# Autodesk Inventor assembly: Assembly
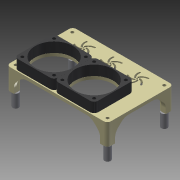
[picture p0: Inventor's stored thumbnail of the model, 180x180]
Saved by Autodesk Inventor 2014 (Build 180170000, 170)
## iProperties
Created: 2017-03-01
Part Number: Assembly
Document SubType Name: Assembly
Designer: Rubén
Author: Rubén
## Documents named in this file (4)
- C:\Users\Rubén\Documents\GitHub\my-3D-printing-designs\Prusa i3 Steel parts\SAV case\Version #2\Assembly.iam
- C:\Users\Rubén\Documents\GitHub\my-3D-printing-designs\Prusa i3 Steel parts\SAV case\Version #2\SAV case.ipt
- C:\Users\Rubén\Documents\GitHub\my-3D-printing-designs\Prusa i3 Steel parts\SAV case\Version #2\Fan 4x4.ipt
- C:\Users\Rubén\Documents\GitHub\my-3D-printing-designs\Prusa i3 Steel parts\SAV case\Version #2\SAV separator.ipt
## Components (7 placed, 3 different names)
1. SAV case:1 — Mate:1, Mate:2, Mate:3, Mate:4, Mate:5, Mate:6, Mate:7, Mate:8, Mate:9, Mate:10, Mate:11, Mate:12, Mate:13, Mate:14
2. Fan 4x4:1 — Mate:4, Mate:5, Mate:6
3. Fan 4x4:2 — Mate:1, Mate:2, Mate:3
4. SAV separator:1 — Mate:7, Mate:11
5. SAV separator:2 — Mate:9, Mate:13
6. SAV separator:3 — Mate:8, Mate:14
7. SAV separator:4 — Mate:10, Mate:12
## Relationships (14: Mate 14)
- Mate:1: SAV case:1 ↔ Fan 4x4:2
- Mate:2: SAV case:1 ↔ Fan 4x4:2
- Mate:3: SAV case:1 ↔ Fan 4x4:2
- Mate:4: SAV case:1 ↔ Fan 4x4:1
- Mate:5: SAV case:1 ↔ Fan 4x4:1
- Mate:6: SAV case:1 ↔ Fan 4x4:1
- Mate:7: SAV case:1 ↔ SAV separator:1
- Mate:8: SAV case:1 ↔ SAV separator:3
- Mate:9: SAV case:1 ↔ SAV separator:2
- Mate:10: SAV case:1 ↔ SAV separator:4
- Mate:11 (1.6 mm): SAV case:1 ↔ SAV separator:1
- Mate:12 (1.6 mm): SAV case:1 ↔ SAV separator:4
- Mate:13 (1.6 mm): SAV case:1 ↔ SAV separator:2
- Mate:14 (1.6 mm): SAV case:1 ↔ SAV separator:3
